# Autodesk Inventor assembly: ASY HPR 340 Feeder head
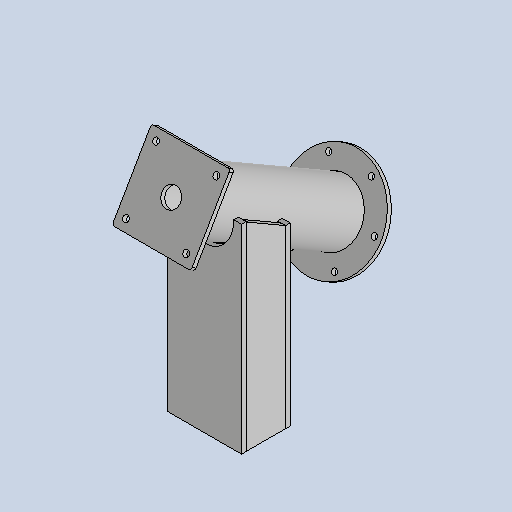
[picture p0: Inventor's stored thumbnail of the model, 512x512]
Saved by Autodesk Inventor 2025.1 (Build 291241020, 241B)
## iProperties
Created: 2024-12-06
Part Number: ASY HPR 340 Feeder head
Document SubType Name: Assembly
Designer: user
Author: user
## Documents named in this file (7)
- C:\Users\user\YandexDisk-badmisterfox\домашниий пк\Inventor\NDM-VOS_powder_hopper\ASY HPR 600 Feeder head.iam
- C:\Users\user\YandexDisk-badmisterfox\домашниий пк\Inventor\NDM-VOS_powder_hopper\NVPH-404 second tube.ipt
- C:\Users\user\YandexDisk-badmisterfox\домашниий пк\Inventor\NDM-VOS_powder_hopper\NVPH-402 tube flange 1.ipt
- C:\Users\user\YandexDisk-badmisterfox\домашниий пк\Inventor\NDM-VOS_powder_hopper\NVPH-412 cup head flange.ipt
- C:\Users\user\YandexDisk-badmisterfox\домашниий пк\Inventor\NDM-VOS_powder_hopper\NVPH-408 feeder hose 1.ipt
- C:\Users\user\YandexDisk-badmisterfox\домашниий пк\Inventor\NDM-VOS_powder_hopper\NVPH-409 feeder hose 2.ipt
- C:\Users\user\YandexDisk-badmisterfox\домашниий пк\Inventor\NDM-VOS_powder_hopper\NVPH-410 feeder hose 3.ipt
## Components (7 placed, 6 different names)
1. NVPH-404 second tube:1 — Rotational:2, Mate:1, Mate:2, Rigid:3, Rigid:7
2. NVPH-402 tube flange 1:1 — Rotational:2, Flush:1
3. NVPH-412 cup head flange:1 — Rigid:7
4. NVPH-408 feeder hose 1:1 — Rigid:3, Rigid:4, Rigid:5, Rigid:6
5. NVPH-409 feeder hose 2:1 — Rigid:4
6. NVPH-410 feeder hose 3:1 — Rigid:5
7. NVPH-410 feeder hose 3:2 — Rigid:6
## Relationships (9: WeldJoint 5, Mate 2, RevoluteJoint 1, Flush 1)
- Rotational:2 [RevoluteJoint]: NVPH-404 second tube:1 ↔ NVPH-402 tube flange 1:1
- Mate:1: NVPH-404 second tube:1
- Flush:1: NVPH-402 tube flange 1:1
- Mate:2: NVPH-404 second tube:1
- Rigid:3 [WeldJoint]: NVPH-404 second tube:1 ↔ NVPH-408 feeder hose 1:1
- Rigid:4 [WeldJoint] (85 mm): NVPH-408 feeder hose 1:1 ↔ NVPH-409 feeder hose 2:1
- Rigid:5 [WeldJoint]: NVPH-408 feeder hose 1:1 ↔ NVPH-410 feeder hose 3:1
- Rigid:6 [WeldJoint]: NVPH-408 feeder hose 1:1 ↔ NVPH-410 feeder hose 3:2
- Rigid:7 [WeldJoint]: NVPH-404 second tube:1 ↔ NVPH-412 cup head flange:1
